# Autodesk Inventor assembly: assembly down part
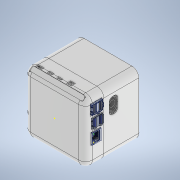
[picture p0: Inventor's stored thumbnail of the model, 180x180]
Saved by Autodesk Inventor 2022.2 (Build 262287010, 287A)
## iProperties
Created: 2022-02-22
Part Number: assembly down part
Document SubType Name: Assembly
Designer: ONG
Author: ONG
## Documents named in this file (14)
- C:\Users\ONG\Documents\INVENTOR DESIGN\音箱\total assembly.iam
- C:\Users\ONG\Documents\INVENTOR DESIGN\音箱\Part3.ipt
- C:\Users\ONG\Downloads\raspeberry pi 4\Raspberry Pi 4 Model B.iam
- C:\Users\ONG\Documents\INVENTOR DESIGN\音箱\part 4.ipt
- C:\Users\ONG\Documents\INVENTOR DESIGN\音箱\speaker stand assembly.iam
- C:\Users\ONG\Documents\INVENTOR DESIGN\音箱\cover.ipt
- C:\Users\ONG\Documents\INVENTOR DESIGN\音箱\assrmbly camera.iam
- C:\Users\ONG\Documents\INVENTOR DESIGN\音箱\assembly down part\Design Accelerator\Bolted Connection1.iam
- C:\Users\ONG\Documents\INVENTOR DESIGN\音箱\assembly down part\Design Accelerator\Bolted Connection3.iam
- C:\Users\ONG\Documents\INVENTOR DESIGN\音箱\assembly down part\Design Accelerator\Bolted Connection4.iam
- C:\Users\ONG\Documents\INVENTOR DESIGN\音箱\assembly down part\Design Accelerator\Bolted Connection5.iam
- C:\Users\ONG\Documents\INVENTOR DESIGN\音箱\assembly down part\Design Accelerator\Bolted Connection7.iam
- C:\Users\ONG\Documents\INVENTOR DESIGN\音箱\assembly down part\Design Accelerator\Bolted Connection8.iam
- C:\Users\ONG\Documents\INVENTOR DESIGN\音箱\assembly down part\Design Accelerator\Bolted Connection9.iam
## Components (14 placed, 7 different names)
1. Part3:1 — Mate:1, Mate:2, Mate:3, Mate:4, Flush:1, Flush:2
2. Raspberry Pi 4 Model B:1 [sub-assembly] — Mate:1, Mate:2, Mate:3, Mate:18, Mate:19
3. part 4:1 — Mate:4, Flush:1, Flush:2, Mate:5, Mate:6, Mate:7, Mate:8, Mate:9, Mate:10, Mate:11, Mate:12, Mate:13, Flush:3, Flush:4, Mate:22, Mate:23
4. speaker stand assembly:1 [sub-assembly] — Mate:5, Mate:6, Mate:7, Mate:14, Mate:15, Mate:26, Mate:27, Mate:32, Mate:33
5. speaker stand assembly:2 [sub-assembly] — Mate:8, Mate:9, Mate:10, Mate:24, Mate:25
6. cover:1 — Mate:11, Mate:12, Mate:13, Insert:1, Mate:30, Mate:31
7. assrmbly camera:1 [sub-assembly] — Insert:1
8. Bolted Connection:1 [sub-assembly] — Mate:14, Mate:15
9. Bolted Connection:2 [sub-assembly] — Mate:32, Mate:33
10. Bolted Connection:3 [sub-assembly] — Mate:18, Mate:19
11. Bolted Connection:4 [sub-assembly] — Mate:22, Mate:23
12. Bolted Connection:5 [sub-assembly] — Mate:24, Mate:25
13. Bolted Connection:6 [sub-assembly] — Mate:26, Mate:27
14. Bolted Connection:7 [sub-assembly] — Mate:30, Mate:31
## Relationships (32: Mate 27, Flush 4, Insert 1)
- Mate:1 (5 mm): Part3:1 ↔ Raspberry Pi 4 Model B:1
- Mate:2: Part3:1 ↔ Raspberry Pi 4 Model B:1
- Mate:3 (2 mm): Part3:1 ↔ Raspberry Pi 4 Model B:1
- Mate:4: Part3:1 ↔ part 4:1
- Flush:1: Part3:1 ↔ part 4:1
- Flush:2: Part3:1 ↔ part 4:1
- Mate:5: part 4:1 ↔ speaker stand assembly:1
- Mate:6: part 4:1 ↔ speaker stand assembly:1
- Mate:7 (20 mm): part 4:1 ↔ speaker stand assembly:1
- Mate:8: part 4:1 ↔ speaker stand assembly:2
- Mate:9: part 4:1 ↔ speaker stand assembly:2
- Mate:10 (5 mm): part 4:1 ↔ speaker stand assembly:2
- Mate:11: part 4:1 ↔ cover:1
- Mate:12: part 4:1 ↔ cover:1
- Mate:13: part 4:1 ↔ cover:1
- Flush:3 (-2 mm): part 4:1
- Flush:4: part 4:1
- Insert:1 (-12 mm): cover:1 ↔ assrmbly camera:1
- Mate:14: speaker stand assembly:1 ↔ Bolted Connection:1
- Mate:15: speaker stand assembly:1 ↔ Bolted Connection:1
- Mate:18: Raspberry Pi 4 Model B:1 ↔ Bolted Connection:3
- Mate:19: Raspberry Pi 4 Model B:1 ↔ Bolted Connection:3
- Mate:22: part 4:1 ↔ Bolted Connection:4
- Mate:23: part 4:1 ↔ Bolted Connection:4
- Mate:24: speaker stand assembly:2 ↔ Bolted Connection:5
- Mate:25: speaker stand assembly:2 ↔ Bolted Connection:5
- Mate:26: speaker stand assembly:1 ↔ Bolted Connection:6
- Mate:27: speaker stand assembly:1 ↔ Bolted Connection:6
- Mate:30: cover:1 ↔ Bolted Connection:7
- Mate:31: cover:1 ↔ Bolted Connection:7
- Mate:32: speaker stand assembly:1 ↔ Bolted Connection:2
- Mate:33: speaker stand assembly:1 ↔ Bolted Connection:2
